# Autodesk Inventor assembly: intake_gearbox_mirrored
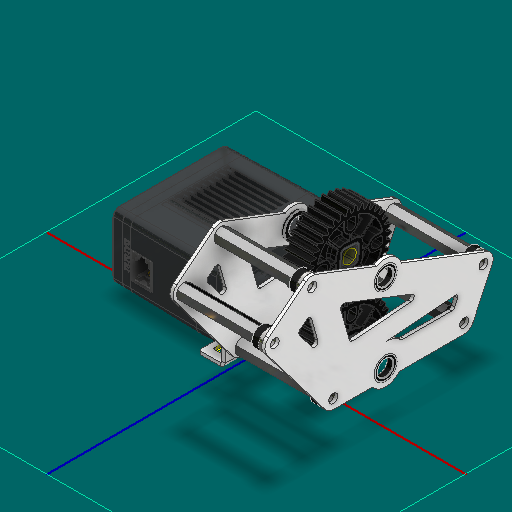
[picture p0: Inventor's stored thumbnail of the model, 512x512]
Saved by Autodesk Inventor 2025 (Build 290162000, 162)
## iProperties
Created: 2024-07-02
Part Number: intake_gearbox_mirrored
Document SubType Name: Assembly
Designer: Averey Ku
Author: Averey Ku
## Documents named in this file (13)
- C:\Users\avere\vex_robotics_high_stakes\hardware\cad\EARLY_SEASON\tower\mirored_parts\intake_gearbox_mirrored.iam
- C:\Users\avere\vex_robotics_high_stakes\hardware\cad\EARLY_SEASON\tower\mirored_parts\HS 36T Gear, No Insert_mirrored.iam
- C:\Users\avere\vex_robotics_high_stakes\hardware\cad\EARLY_SEASON\tower\mirored_parts\Alu Angle 1x1x6_mirrored.ipt
- C:\Users\avere\vex_robotics_high_stakes\hardware\cad\EARLY_SEASON\tower\mirored_parts\gearbox_gusset_mirrored.ipt
- C:\Users\avere\vex_robotics_high_stakes\hardware\cad\EARLY_SEASON\tower\mirored_parts\HS Bushing 0.1250_mirrored.ipt
- C:\Users\avere\vex_robotics_high_stakes\hardware\cad\EARLY_SEASON\tower\mirored_parts\V5 Motor_mirrored.ipt
- C:\Users\avere\vex_robotics_high_stakes\hardware\cad\EARLY_SEASON\tower\mirored_parts\6P 8T Sprocket, No Insert_mirrored.iam
- C:\Users\avere\vex_robotics_high_stakes\hardware\cad\VEX-CAD-Inventor\Structure\Standoff\Standoff 1.50.ipt
- D:\vex_robotics_high_stakes\hardware\cad\VEX-CAD-Inventor\Structure\Standoff.ipt
- C:\Users\avere\vex_robotics_high_stakes\hardware\cad\VEX-CAD-Inventor\Motion\Spacers\Spacer Nylon .375 OD\NSpacer .375 OD x .125.ipt
- D:\vex_robotics_high_stakes\hardware\cad\VEX-CAD-Inventor\Motion\Spacers\Spacer Nylon .375 OD.ipt
- C:\Users\avere\vex_robotics_high_stakes\hardware\cad\VEX-CAD-Inventor\Motion\Spacers\Washer Steel\SWasher .375 OD x .062500.ipt
- D:\vex_robotics_high_stakes\hardware\cad\VEX-CAD-Inventor\Motion\Spacers\Washer Steel.ipt
## Components (26 placed, 9 different names)
1. HS 36T Gear, No Insert_mirrored:1 [sub-assembly] — Insert:9
2. HS 36T Gear, No Insert_mirrored:2 [sub-assembly] — Insert:7, Insert:10
3. Alu Angle 1x1x6_mirrored:1 — Insert:6, Mate:2, Insert:8, Mate:3
4. gearbox_gusset_mirrored:1 — Insert:5, Mate:1, Insert:2, Insert:3
5. gearbox_gusset_mirrored:2 — Insert:5, Insert:6, Mate:2, Mate:1, Insert:1, Insert:4, Insert:11, Insert:12, Insert:13, Insert:14, Insert:15
6. HS Bushing 0.1250_mirrored:1 — Insert:7, Insert:1
7. HS Bushing 0.1250_mirrored:2 — Insert:2
8. HS Bushing 0.1250_mirrored:3 — Insert:3
9. HS Bushing 0.1250_mirrored:4 — Insert:9, Insert:4
10. V5 Motor_mirrored:1 — Insert:8, Mate:3
11. 6P 8T Sprocket, No Insert_mirrored:1 [sub-assembly] — Insert:10
12. Standoff 1.50:1 — Insert:11, Insert:22
13. Standoff 1.50:2 — Insert:12, Insert:23
14. Standoff 1.50:3 — Insert:13, Insert:20
15. Standoff 1.50:4 — Insert:14, Insert:21
16. Standoff 1.50:5 — Insert:15, Insert:25
17. NSpacer .375 OD x .125:1 — Insert:22, Insert:17
18. NSpacer .375 OD x .125:2 — Insert:20, Insert:19
19. NSpacer .375 OD x .125:3 — Insert:21, Insert:16
20. NSpacer .375 OD x .125:4 — Insert:23, Insert:18
21. SWasher .375 OD x .062500:1 — Insert:18
22. SWasher .375 OD x .062500:2 — Insert:16
23. SWasher .375 OD x .062500:3 — Insert:19
24. SWasher .375 OD x .062500:4 — Insert:17
25. NSpacer .375 OD x .125:5 — Insert:25, Insert:24
26. SWasher .375 OD x .062500:5 — Insert:24
## Relationships (28: Insert 25, Mate 3)
- Insert:5 (42.8625 mm): gearbox_gusset_mirrored:1 ↔ gearbox_gusset_mirrored:2
- Insert:6: Alu Angle 1x1x6_mirrored:1 ↔ gearbox_gusset_mirrored:2
- Mate:2: Alu Angle 1x1x6_mirrored:1 ↔ gearbox_gusset_mirrored:2
- Mate:1: gearbox_gusset_mirrored:1 ↔ gearbox_gusset_mirrored:2
- Insert:7 (12.7 mm): HS 36T Gear, No Insert_mirrored:2 ↔ HS Bushing 0.1250_mirrored:1
- Insert:1: gearbox_gusset_mirrored:2 ↔ HS Bushing 0.1250_mirrored:1
- Insert:2: gearbox_gusset_mirrored:1 ↔ HS Bushing 0.1250_mirrored:2
- Insert:3: gearbox_gusset_mirrored:1 ↔ HS Bushing 0.1250_mirrored:3
- Insert:9 (12.7 mm): HS 36T Gear, No Insert_mirrored:1 ↔ HS Bushing 0.1250_mirrored:4
- Insert:4: gearbox_gusset_mirrored:2 ↔ HS Bushing 0.1250_mirrored:4
- Insert:8: Alu Angle 1x1x6_mirrored:1 ↔ V5 Motor_mirrored:1
- Mate:3: Alu Angle 1x1x6_mirrored:1 ↔ V5 Motor_mirrored:1
- Insert:10: HS 36T Gear, No Insert_mirrored:2 ↔ 6P 8T Sprocket, No Insert_mirrored:1
- Insert:11: gearbox_gusset_mirrored:2 ↔ Standoff 1.50:1
- Insert:12: gearbox_gusset_mirrored:2 ↔ Standoff 1.50:2
- Insert:13: gearbox_gusset_mirrored:2 ↔ Standoff 1.50:3
- Insert:14: gearbox_gusset_mirrored:2 ↔ Standoff 1.50:4
- Insert:15: gearbox_gusset_mirrored:2 ↔ Standoff 1.50:5
- Insert:22: Standoff 1.50:1 ↔ NSpacer .375 OD x .125:1
- Insert:20: Standoff 1.50:3 ↔ NSpacer .375 OD x .125:2
- Insert:21: Standoff 1.50:4 ↔ NSpacer .375 OD x .125:3
- Insert:23: Standoff 1.50:2 ↔ NSpacer .375 OD x .125:4
- Insert:18: NSpacer .375 OD x .125:4 ↔ SWasher .375 OD x .062500:1
- Insert:16: NSpacer .375 OD x .125:3 ↔ SWasher .375 OD x .062500:2
- Insert:19: NSpacer .375 OD x .125:2 ↔ SWasher .375 OD x .062500:3
- Insert:17: NSpacer .375 OD x .125:1 ↔ SWasher .375 OD x .062500:4
- Insert:25: Standoff 1.50:5 ↔ NSpacer .375 OD x .125:5
- Insert:24: NSpacer .375 OD x .125:5 ↔ SWasher .375 OD x .062500:5
